# Autodesk Inventor assembly: 0005-10-04 Y axis and extruder
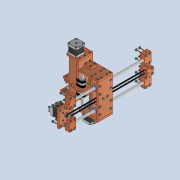
[picture p0: Inventor's stored thumbnail of the model, 180x180]
Saved by Autodesk Inventor 2020 (Build 240168000, 168)
## iProperties
Created: 2020-12-18
Part Number: 0005-10-04 Y axis and extruder
Document SubType Name: Assembly
Designer: Iulian Bors
Mass: 17144.8 g
Surface Area: 27601.7 cm^2
Volume: 16303.9 cm^3
Density: 1.05157 g/cm^3
Author: Iulian Bors
## iProperties of the stored document Part 1.ipt
Created: 2020-12-18
Part Number: Part 1
Material: Generic
Document SubType Name: Modeling
Designer: Iulian Bors
Density: 1 g/cm^3
Appearance: Default
Mass: 0.27605 g
Surface Area: 6.48852 cm^2
Volume: 0.27605 cm^3
Author: Iulian Bors
Revision Number: NONE
## iProperties of the stored document Part 2.ipt
Created: 2020-12-18
Part Number: Part 2
Material: Generic
Document SubType Name: Modeling
Designer: Iulian Bors
Density: 1 g/cm^3
Appearance: Default
Mass: 0.0253291 g
Surface Area: 2.0565 cm^2
Volume: 0.0253291 cm^3
Author: Iulian Bors
Revision Number: NONE
## iProperties of the stored document Needle.iam
Created: 2020-01-23
Part Number: Needle
Document SubType Name: Assembly
Designer: Iulian Bors
Mass: 0.301379 g
Surface Area: 8.54503 cm^2
Volume: 0.301379 cm^3
Density: 1 g/cm^3
Title: /vol/tmp/translate-4006329005178005204/5e293bbb2de6b7156cc2e2d4.step
## Documents named in this file (37)
- Z:\I.A.B\Proiecte\0005 I.A.B 3d 2.0 Imprimanta aracet\10 Mecanic\0005-10-04 Y axis and extruder.iam
- Z:\I.A.B\Proiecte\0005 I.A.B 3d 2.0 Imprimanta aracet\10 Mecanic\Seringa\body 20ml_Défaut.ipt
- Z:\I.A.B\Proiecte\0005 I.A.B 3d 2.0 Imprimanta aracet\10 Mecanic\Seringa\Plunger Assembly_Défaut.iam
- **Z:\I.A.B\Proiecte\0005 I.A.B 3d 2.0 Imprimanta aracet\10 Mecanic\0005-10-04 Y axis and extruder.iam*LocalDocs*xAaaaqeaaAaaaaaaaAaaaq3zaLd*Needle.iam
- Z:\I.A.B\Proiecte\0005 I.A.B 3d 2.0 Imprimanta aracet\10 Mecanic\0005-10-003 Actionare seringa.ipt
- Z:\I.A.B\Proiecte\0005 I.A.B 3d 2.0 Imprimanta aracet\10 Mecanic\0005-10-004 Actionare 2 seringa.ipt
- Z:\I.A.B\Proiecte\0005 I.A.B 3d 2.0 Imprimanta aracet\10 Mecanic\0005-10-1004 Piulita.ipt
- Z:\I.A.B\Proiecte\0005 I.A.B 3d 2.0 Imprimanta aracet\10 Mecanic\0005-10-10-1003 LeadScrew 8mm x 2mmPitch.ipt
- Z:\I.A.B\Proiecte\0005 I.A.B 3d 2.0 Imprimanta aracet\10 Mecanic\0005-10-1005 ISO 1224-1 - 10 - 8 x 22 x 7.ipt
- Z:\I.A.B\Proiecte\0005 I.A.B 3d 2.0 Imprimanta aracet\10 Mecanic\0005-10-005.ipt
- Z:\I.A.B\Proiecte\0005 I.A.B 3d 2.0 Imprimanta aracet\10 Mecanic\0005-10-006 Capac rulment.ipt
- Z:\I.A.B\Proiecte\0005 I.A.B 3d 2.0 Imprimanta aracet\10 Mecanic\0005-10-1002  Hub.ipt
- Z:\I.A.B\Proiecte\0005 I.A.B 3d 2.0 Imprimanta aracet\10 Mecanic\0005-10-1001 NEMA17 - Motor de passo.ipt
- Z:\I.A.B\Proiecte\0005 I.A.B 3d 2.0 Imprimanta aracet\10 Mecanic\0005-10-007Suport nema.ipt
- Z:\I.A.B\Proiecte\0005 I.A.B 3d 2.0 Imprimanta aracet\10 Mecanic\0005-10-008.ipt
- Z:\I.A.B\Proiecte\0005 I.A.B 3d 2.0 Imprimanta aracet\10 Mecanic\0005-10-009.ipt
- Z:\I.A.B\Proiecte\0005 I.A.B 3d 2.0 Imprimanta aracet\10 Mecanic\0005-10-010.ipt
- Z:\I.A.B\Proiecte\0005 I.A.B 3d 2.0 Imprimanta aracet\10 Mecanic\0005-10-1006 Bara rectificata.ipt
- Z:\I.A.B\Proiecte\0005 I.A.B 3d 2.0 Imprimanta aracet\10 Mecanic\0005-10-1009 LM10uu.ipt
- Z:\I.A.B\Proiecte\0005 I.A.B 3d 2.0 Imprimanta aracet\10 Mecanic\0005-10-002 Suport1 Seringa.ipt
- Z:\I.A.B\Proiecte\0005 I.A.B 3d 2.0 Imprimanta aracet\10 Mecanic\0005-10-016.ipt
- Z:\I.A.B\Proiecte\0005 I.A.B 3d 2.0 Imprimanta aracet\10 Mecanic\0005-10-021 suport senzor z.ipt
- Z:\I.A.B\Proiecte\0005 I.A.B 3d 2.0 Imprimanta aracet\10 Mecanic\0005-10-1000 LM8.ipt
- Z:\I.A.B\Proiecte\0005 I.A.B 3d 2.0 Imprimanta aracet\10 Mecanic\0005-10-1018 tija 8.ipt
- Z:\I.A.B\Proiecte\0005 I.A.B 3d 2.0 Imprimanta aracet\10 Mecanic\Surub M3 40 mm.iam
- Z:\I.A.B\Proiecte\0005 I.A.B 3d 2.0 Imprimanta aracet\10 Mecanic\0005-10-1020 ISO 7089 - 3 - 140 HV(1).ipt
- Z:\I.A.B\Proiecte\0005 I.A.B 3d 2.0 Imprimanta aracet\10 Mecanic\0005-10-01 Cadru.iam
- Z:\I.A.B\Proiecte\0005 I.A.B 3d 2.0 Imprimanta aracet\10 Mecanic\0005-10-02 X axis.iam
- Z:\I.A.B\Proiecte\0005 I.A.B 3d 2.0 Imprimanta aracet\10 Mecanic\0005-10-1032.ipt
- Z:\I.A.B\Proiecte\0005 I.A.B 3d 2.0 Imprimanta aracet\10 Mecanic\Surub M3 25.iam
- Z:\I.A.B\Proiecte\0005 I.A.B 3d 2.0 Imprimanta aracet\10 Mecanic\0005-10-1021 ISO 4032 - M3 - ISO.ipt
- Z:\I.A.B\Proiecte\0005 I.A.B 3d 2.0 Imprimanta aracet\10 Mecanic\Colier.ipt
- C:\Users\40743\Documents\Inventor\Content Center Files\R2020\en-US\ISO 7050 - C-Z(2)\ISO 7050 - ST 3.5 x 22 - C - Z.ipt
- **Z:\I.A.B\Proiecte\0005 I.A.B 3d 2.0 Imprimanta aracet\0005-00-00 Ansamblu_General.iam*LocalDocs*xAaaaaecaAaaaaaaaAaaaqfy1Od*Part 1.ipt
- **Z:\I.A.B\Proiecte\0005 I.A.B 3d 2.0 Imprimanta aracet\0005-00-00 Ansamblu_General.iam*LocalDocs*xAaaaa4baAaaaaaaaAaaaq4bsZa*Part 2.ipt
- **Z:\I.A.B\Proiecte\0005 I.A.B 3d 2.0 Imprimanta aracet\0005-00-00 Ansamblu_General.iam*LocalDocs*xAaaaqeaaAaaaaaaaAaaaq3zaLd*Needle.iam
- Z:\I.A.B\Proiecte\0005 I.A.B 3d 2.0 Imprimanta aracet\10 Mecanic\Seringa\21-gauge-needle-1.snapshot.2\Needle.step
## Components (93 placed, 33 different names)
1. Needle.iam:4 [sub-assembly] — Insert:14
2. 0005-10-10-1003 LeadScrew 8mm x 2mmPitch.ipt:5 — Insert:2, Insert:4, Mate:61, Mate:118
3. 0005-10-1005 ISO 1224-1 - 10 - 8 x 22 x 7.ipt:6 — Insert:2, Mate:15, Insert:3
4. 0005-10-005.ipt:7 — Mate:15, Mate:16, Flush:4, Mate:17, Flush:76, Flush:7, Mate:50, Mate:51, Angle:9, Mate:59, Mate:61, Flush:35, Mate:137, Mate:138, Mate:142, Insert:67, Insert:68, Insert:76, Insert:77, Insert:78
5. 0005-10-006 Capac rulment.ipt:8 — Insert:3, Insert:62, Insert:63, Insert:64, Mate:142, Mate:143
6. 0005-10-1002  Hub.ipt:9 — Insert:4, Insert:5
7. 0005-10-1001 NEMA17 - Motor de passo.ipt:10 — Insert:5, Angle:14
8. 0005-10-008.ipt:11 — Mate:16, Flush:4, Flush:11, Mate:21, Angle:11, Mate:158, Mate:159
9. 0005-10-008.ipt:12 — Mate:17, Flush:7, Mate:119, Flush:64, Angle:16, Mate:157
10. 0005-10-016.ipt:13 — Flush:76, Mate:19, Mate:20, Flush:18, Flush:35, Flush:63
11. 0005-10-009.ipt:14 — Mate:19, Flush:11, Flush:18, Flush:63, Flush:65, Angle:15, Mate:157, Mate:158
12. 0005-10-010.ipt:15 — Mate:20, Mate:21, Insert:7, Mate:35, Mate:37, Mate:103, Insert:26, Insert:27, Mate:147, Mate:150, Mate:153, Mate:155, Mate:159
13. 0005-10-1004 Piulita.ipt:16 — Mate:35, Mate:36
14. 0005-10-1009 LM10uu.ipt:17 — Insert:7, Mate:26, Flush:57, Mate:145, Mate:146
15. 0005-10-1006 Bara rectificata.ipt:18 — Mate:26, Insert:41
16. 0005-10-1006 Bara rectificata.ipt:19 — Mate:103, Mate:104, Insert:42
17. 0005-10-10-1003 LeadScrew 8mm x 2mmPitch.ipt:21 — Mate:33, Mate:36, Mate:37, Insert:37, Insert:38
18. 0005-10-1002  Hub.ipt:22 — Mate:33
19. 0005-10-1001 NEMA17 - Motor de passo.ipt:23 — Insert:37, Mate:139, Angle:13
20. 0005-10-006 Capac rulment.ipt:26 — Insert:39, Mate:141
21. 0005-10-1005 ISO 1224-1 - 10 - 8 x 22 x 7.ipt:27 — Insert:38, Insert:39
22. 0005-10-1004 Piulita.ipt:38 — Insert:13, Mate:140, Insert:72
23. body 20ml_Défaut.ipt:39 — Mate:50, Mate:51, Angle:9, Mate:52, Insert:14
24. Plunger Assembly_Défaut.iam:40 [sub-assembly] — Mate:52, Mate:53
25. 0005-10-003 Actionare seringa.ipt:41 — Insert:13, Mate:53, Angle:11, Mate:117, Mate:118, Insert:22, Mate:121, Mate:122, Mate:140, Insert:65, Insert:66
26. 0005-10-004 Actionare 2 seringa.ipt:42 — Insert:22, Mate:122
27. 0005-10-002 Suport1 Seringa.ipt:43 — Mate:59, Mate:137, Mate:138
28. 0005-10-021 suport senzor z.ipt:75 — Mate:144
29. 0005-10-1009 LM10uu.ipt:79 — Mate:104, Flush:57, Mate:151, Flush:71, Mate:152
30. 0005-10-1000 LM8.ipt:85 — Mate:117, Mate:120
31. 0005-10-007Suport nema.ipt:86 — Mate:119, Flush:64, Flush:65, Flush:66, Angle:14, Insert:55, Insert:56, Insert:57, Insert:73, Insert:74, Insert:75
32. 0005-10-1018 tija 8.ipt:87 — Mate:120, Mate:121, Flush:66
33. Surub M3 40 mm.iam:89 [sub-assembly] — Insert:43
34. 0005-10-1009 LM10uu.ipt:91 — Insert:27, Mate:148, Flush:68, Mate:149
35. 0005-10-1009 LM10uu.ipt:92 — Insert:26, Mate:154, Mate:156, Flush:74
36. 0005-10-01 Cadru:1 [sub-assembly] — Insert:40
37. 0005-10-02 X axis:1 [sub-assembly] — Insert:40, Angle:12, Insert:41, Insert:42, Mate:139, Angle:13, Insert:43, Mate:141, Insert:44, Insert:45, Insert:46, Insert:58, Insert:59, Insert:60, Insert:61, Mate:144
38. Surub M3 40 mm:2 [sub-assembly] — Insert:44
39. Surub M3 40 mm:3 [sub-assembly] — Insert:45
40. Surub M3 40 mm:4 [sub-assembly] — Insert:46
41. DIN 7984 M3 x 16:1
42. ISO 7089 3:2 — Insert:55
43. DIN 7984 M3 x 16:2
44. ISO 7089 3:3 — Insert:58
45. DIN 7984 M3 x 16:4
46. ISO 7089 3:5 — Insert:57
47. DIN 7984 M3 x 16:5
48. ISO 7089 3:6 — Insert:61
49. DIN 7984 M3 x 16:6
50. ISO 7089 3:7 — Insert:59
51. DIN 7984 M3 x 16:7
52. ISO 7089 3:8 — Insert:60
53. DIN 7984 M3 x 16:8
54. ISO 7089 3:9 — Insert:56
55. Surub M3 40 mm:5 [sub-assembly] — Insert:64
56. Surub M3 40 mm:6 [sub-assembly] — Insert:63
57. Surub M3 40 mm:7 [sub-assembly] — Insert:62
58. Surub M3 40 mm:8 [sub-assembly] — Mate:143
59. Surub M3 25:1 [sub-assembly] — Insert:65
60. Surub M3 25:2 [sub-assembly] — Insert:66
61. Surub M3 25:3 [sub-assembly] — Insert:67
62. Surub M3 25:4 [sub-assembly] — Insert:68
63. Colier:1 — Mate:145, Angle:15, Flush:67
64. Colier:2 — Mate:146, Mate:147, Flush:67, Flush:69, Flush:70
65. Colier:3 — Mate:148, Flush:68, Flush:69
66. Colier:4 — Mate:149, Mate:150, Flush:70
67. Colier:5 — Mate:151, Angle:16, Flush:71, Flush:72
68. Colier:6 — Mate:152, Mate:153, Flush:72, Flush:73
69. Colier:7 — Mate:154, Mate:155, Flush:73, Flush:75
70. Colier:8 — Mate:156, Flush:74, Flush:75
71. ISO 7050 - C-Z ST 3.5 x 22 - C - Z:1 — Insert:73
72. ISO 7050 - C-Z ST 3.5 x 22 - C - Z:2 — Insert:76
73. ISO 7050 - C-Z ST 3.5 x 22 - C - Z:3 — Insert:78
74. ISO 7050 - C-Z ST 3.5 x 22 - C - Z:4 — Insert:74
75. ISO 7050 - C-Z ST 3.5 x 22 - C - Z:5 — Insert:75
76. ISO 7050 - C-Z ST 3.5 x 22 - C - Z:6 — Insert:77
77. ISO 7050 - C-Z ST 3.5 x 22 - C - Z:7
78. DIN 7984 M3 x 16:9 — Insert:70
79. ISO 7089 3:10 — Insert:72
80. ISO 4032 M3:1 — Insert:70, Insert:71
81. ISO 7089 3:11 — Insert:71
82. DIN 7984 M3 x 16:10
83. ISO 7089 3:12
84. ISO 4032 M3:2
85. ISO 7089 3:13
86. DIN 7984 M3 x 16:11
87. ISO 7089 3:14
88. ISO 4032 M3:3
89. ISO 7089 3:15
90. DIN 7984 M3 x 16:12
91. ISO 7089 3:16
92. ISO 4032 M3:4
93. ISO 7089 3:17
## Component patterns: (4 elements, first: DIN 7984 M3 x 16:9 + ISO 7089 3:10 + ISO 4032 M3:1 + ISO 7089 3:11)
## Relationships (127: Insert 52, Mate 48, Flush 20, Angle 7)
- Insert:2: 0005-10-10-1003 LeadScrew 8mm x 2mmPitch.ipt:5 ↔ 0005-10-1005 ISO 1224-1 - 10 - 8 x 22 x 7.ipt:6
- Mate:15: 0005-10-1005 ISO 1224-1 - 10 - 8 x 22 x 7.ipt:6 ↔ 0005-10-005.ipt:7
- Insert:3: 0005-10-1005 ISO 1224-1 - 10 - 8 x 22 x 7.ipt:6 ↔ 0005-10-006 Capac rulment.ipt:8
- Insert:4: 0005-10-10-1003 LeadScrew 8mm x 2mmPitch.ipt:5 ↔ 0005-10-1002  Hub.ipt:9
- Insert:5 (5 mm): 0005-10-1002  Hub.ipt:9 ↔ 0005-10-1001 NEMA17 - Motor de passo.ipt:10
- Mate:16: 0005-10-005.ipt:7 ↔ 0005-10-008.ipt:11
- Flush:4: 0005-10-005.ipt:7 ↔ 0005-10-008.ipt:11
- Mate:17: 0005-10-005.ipt:7 ↔ 0005-10-008.ipt:12
- Flush:76: 0005-10-005.ipt:7 ↔ 0005-10-016.ipt:13
- Flush:7: 0005-10-005.ipt:7 ↔ 0005-10-008.ipt:12
- Mate:19 (8 mm): 0005-10-016.ipt:13 ↔ 0005-10-009.ipt:14
- Flush:11: 0005-10-008.ipt:11 ↔ 0005-10-009.ipt:14
- Mate:20: 0005-10-016.ipt:13 ↔ 0005-10-010.ipt:15
- Mate:21: 0005-10-008.ipt:11 ↔ 0005-10-010.ipt:15
- Insert:7: 0005-10-010.ipt:15 ↔ 0005-10-1009 LM10uu.ipt:17
- Mate:26: 0005-10-1009 LM10uu.ipt:17 ↔ 0005-10-1006 Bara rectificata.ipt:18
- [Insert] (5 mm): 0005-10-1002  Hub.ipt:22 ↔ 0005-10-1001 NEMA17 - Motor de passo.ipt:23
- Mate:33: 0005-10-10-1003 LeadScrew 8mm x 2mmPitch.ipt:21 ↔ 0005-10-1002  Hub.ipt:22
- Mate:35: 0005-10-010.ipt:15 ↔ 0005-10-1004 Piulita.ipt:16
- Mate:36: 0005-10-1004 Piulita.ipt:16 ↔ 0005-10-10-1003 LeadScrew 8mm x 2mmPitch.ipt:21
- Mate:37: 0005-10-010.ipt:15 ↔ 0005-10-10-1003 LeadScrew 8mm x 2mmPitch.ipt:21
- Flush:18: 0005-10-016.ipt:13 ↔ 0005-10-009.ipt:14
- Mate:50: 0005-10-005.ipt:7 ↔ body 20ml_Défaut.ipt:39
- Mate:51: 0005-10-005.ipt:7 ↔ body 20ml_Défaut.ipt:39
- Angle:9 (0 deg): 0005-10-005.ipt:7 ↔ body 20ml_Défaut.ipt:39
- Mate:52: body 20ml_Défaut.ipt:39 ↔ Plunger Assembly_Défaut.iam:40
- Insert:13: 0005-10-1004 Piulita.ipt:38 ↔ 0005-10-003 Actionare seringa.ipt:41
- Mate:53: Plunger Assembly_Défaut.iam:40 ↔ 0005-10-003 Actionare seringa.ipt:41
- Insert:14 (-5 mm): Needle.iam:4 ↔ body 20ml_Défaut.ipt:39
- Angle:11 (0 deg): 0005-10-008.ipt:11 ↔ 0005-10-003 Actionare seringa.ipt:41
- Mate:59: 0005-10-005.ipt:7 ↔ 0005-10-002 Suport1 Seringa.ipt:43
- Mate:61: 0005-10-10-1003 LeadScrew 8mm x 2mmPitch.ipt:5 ↔ 0005-10-005.ipt:7
- Flush:35 (8 mm): 0005-10-005.ipt:7 ↔ 0005-10-016.ipt:13
- Mate:103: 0005-10-010.ipt:15 ↔ 0005-10-1006 Bara rectificata.ipt:19
- Mate:104: 0005-10-1006 Bara rectificata.ipt:19 ↔ 0005-10-1009 LM10uu.ipt:79
- Flush:57: 0005-10-1009 LM10uu.ipt:17 ↔ 0005-10-1009 LM10uu.ipt:79
- Mate:117 (-10 mm): 0005-10-003 Actionare seringa.ipt:41 ↔ 0005-10-1000 LM8.ipt:85
- Mate:118: 0005-10-10-1003 LeadScrew 8mm x 2mmPitch.ipt:5 ↔ 0005-10-003 Actionare seringa.ipt:41
- Flush:63: 0005-10-016.ipt:13 ↔ 0005-10-009.ipt:14
- Insert:22 (1 mm): 0005-10-003 Actionare seringa.ipt:41 ↔ 0005-10-004 Actionare 2 seringa.ipt:42
- Mate:119: 0005-10-008.ipt:12 ↔ 0005-10-007Suport nema.ipt:86
- Flush:64: 0005-10-008.ipt:12 ↔ 0005-10-007Suport nema.ipt:86
- Flush:65: 0005-10-009.ipt:14 ↔ 0005-10-007Suport nema.ipt:86
- Mate:120: 0005-10-1000 LM8.ipt:85 ↔ 0005-10-1018 tija 8.ipt:87
- Mate:121: 0005-10-003 Actionare seringa.ipt:41 ↔ 0005-10-1018 tija 8.ipt:87
- Flush:66: 0005-10-007Suport nema.ipt:86 ↔ 0005-10-1018 tija 8.ipt:87
- Mate:122: 0005-10-003 Actionare seringa.ipt:41 ↔ 0005-10-004 Actionare 2 seringa.ipt:42
- Insert:26: 0005-10-010.ipt:15 ↔ 0005-10-1009 LM10uu.ipt:92
- Insert:27: 0005-10-010.ipt:15 ↔ 0005-10-1009 LM10uu.ipt:91
- Mate:137: 0005-10-005.ipt:7 ↔ 0005-10-002 Suport1 Seringa.ipt:43
- Mate:138: 0005-10-005.ipt:7 ↔ 0005-10-002 Suport1 Seringa.ipt:43
- Insert:37: 0005-10-10-1003 LeadScrew 8mm x 2mmPitch.ipt:21 ↔ 0005-10-1001 NEMA17 - Motor de passo.ipt:23
- Insert:38: 0005-10-10-1003 LeadScrew 8mm x 2mmPitch.ipt:21 ↔ 0005-10-1005 ISO 1224-1 - 10 - 8 x 22 x 7.ipt:27
- Insert:39: 0005-10-006 Capac rulment.ipt:26 ↔ 0005-10-1005 ISO 1224-1 - 10 - 8 x 22 x 7.ipt:27
- Insert:40: 0005-10-01 Cadru:1 ↔ 0005-10-02 X axis:1
- Angle:12 (0 deg): 0005-10-02 X axis:1
- Insert:41: 0005-10-1006 Bara rectificata.ipt:18 ↔ 0005-10-02 X axis:1
- Insert:42: 0005-10-1006 Bara rectificata.ipt:19 ↔ 0005-10-02 X axis:1
- Mate:139: 0005-10-1001 NEMA17 - Motor de passo.ipt:23 ↔ 0005-10-02 X axis:1
- Angle:13 (0 deg): 0005-10-1001 NEMA17 - Motor de passo.ipt:23 ↔ 0005-10-02 X axis:1
- Angle:14 (0 deg): 0005-10-1001 NEMA17 - Motor de passo.ipt:10 ↔ 0005-10-007Suport nema.ipt:86
- Mate:140: 0005-10-1004 Piulita.ipt:38 ↔ 0005-10-003 Actionare seringa.ipt:41
- Insert:43: Surub M3 40 mm.iam:89 ↔ 0005-10-02 X axis:1
- Mate:141: 0005-10-006 Capac rulment.ipt:26 ↔ 0005-10-02 X axis:1
- Insert:44: 0005-10-02 X axis:1 ↔ Surub M3 40 mm:2
- Insert:45: 0005-10-02 X axis:1 ↔ Surub M3 40 mm:3
- Insert:46: 0005-10-02 X axis:1 ↔ Surub M3 40 mm:4
- [Insert]: DIN 7984 M3 x 16:1 ↔ ISO 7089 3:2
- [Insert]: DIN 7984 M3 x 16:2 ↔ ISO 7089 3:3
- [Insert]: DIN 7984 M3 x 16:4 ↔ ISO 7089 3:5
- [Insert]: DIN 7984 M3 x 16:5 ↔ ISO 7089 3:6
- [Insert]: DIN 7984 M3 x 16:6 ↔ ISO 7089 3:7
- [Insert]: DIN 7984 M3 x 16:7 ↔ ISO 7089 3:8
- [Insert]: DIN 7984 M3 x 16:8 ↔ ISO 7089 3:9
- Insert:55: 0005-10-007Suport nema.ipt:86 ↔ ISO 7089 3:2
- Insert:56: 0005-10-007Suport nema.ipt:86 ↔ ISO 7089 3:9
- Insert:57: 0005-10-007Suport nema.ipt:86 ↔ ISO 7089 3:5
- Insert:58: 0005-10-02 X axis:1 ↔ ISO 7089 3:3
- Insert:59: 0005-10-02 X axis:1 ↔ ISO 7089 3:7
- Insert:60: 0005-10-02 X axis:1 ↔ ISO 7089 3:8
- Insert:61: 0005-10-02 X axis:1 ↔ ISO 7089 3:6
- Insert:62: 0005-10-006 Capac rulment.ipt:8 ↔ Surub M3 40 mm:7
- Insert:63: 0005-10-006 Capac rulment.ipt:8 ↔ Surub M3 40 mm:6
- Insert:64: 0005-10-006 Capac rulment.ipt:8 ↔ Surub M3 40 mm:5
- Mate:142: 0005-10-005.ipt:7 ↔ 0005-10-006 Capac rulment.ipt:8
- Mate:143: 0005-10-006 Capac rulment.ipt:8 ↔ Surub M3 40 mm:8
- Insert:65: 0005-10-003 Actionare seringa.ipt:41 ↔ Surub M3 25:1
- Insert:66: 0005-10-003 Actionare seringa.ipt:41 ↔ Surub M3 25:2
- Insert:67: 0005-10-005.ipt:7 ↔ Surub M3 25:3
- Insert:68: 0005-10-005.ipt:7 ↔ Surub M3 25:4
- Mate:144: 0005-10-021 suport senzor z.ipt:75 ↔ 0005-10-02 X axis:1
- [Insert]: DIN 7984 M3 x 16:9 ↔ ISO 7089 3:10
- Insert:70: DIN 7984 M3 x 16:9 ↔ ISO 4032 M3:1
- Insert:71: ISO 4032 M3:1 ↔ ISO 7089 3:11
- Insert:72: 0005-10-1004 Piulita.ipt:38 ↔ ISO 7089 3:10
- Mate:145: 0005-10-1009 LM10uu.ipt:17 ↔ Colier:1
- Angle:15 (180 deg): 0005-10-009.ipt:14 ↔ Colier:1
- Mate:146: 0005-10-1009 LM10uu.ipt:17 ↔ Colier:2
- Mate:147: 0005-10-010.ipt:15 ↔ Colier:2
- Flush:67: Colier:1 ↔ Colier:2
- Mate:148: 0005-10-1009 LM10uu.ipt:91 ↔ Colier:3
- Flush:68: 0005-10-1009 LM10uu.ipt:91 ↔ Colier:3
- Flush:69: Colier:2 ↔ Colier:3
- Mate:149: 0005-10-1009 LM10uu.ipt:91 ↔ Colier:4
- Mate:150: 0005-10-010.ipt:15 ↔ Colier:4
- Flush:70: Colier:2 ↔ Colier:4
- Mate:151: 0005-10-1009 LM10uu.ipt:79 ↔ Colier:5
- Angle:16 (0 deg): 0005-10-008.ipt:12 ↔ Colier:5
- Flush:71: 0005-10-1009 LM10uu.ipt:79 ↔ Colier:5
- Mate:152: 0005-10-1009 LM10uu.ipt:79 ↔ Colier:6
- Mate:153: 0005-10-010.ipt:15 ↔ Colier:6
- Flush:72: Colier:5 ↔ Colier:6
- Mate:154: 0005-10-1009 LM10uu.ipt:92 ↔ Colier:7
- Mate:155: 0005-10-010.ipt:15 ↔ Colier:7
- Flush:73: Colier:6 ↔ Colier:7
- Mate:156: 0005-10-1009 LM10uu.ipt:92 ↔ Colier:8
- Flush:74: 0005-10-1009 LM10uu.ipt:92 ↔ Colier:8
- Flush:75: Colier:7 ↔ Colier:8
- Mate:157: 0005-10-008.ipt:12 ↔ 0005-10-009.ipt:14
- Mate:158: 0005-10-008.ipt:11 ↔ 0005-10-009.ipt:14
- Mate:159: 0005-10-008.ipt:11 ↔ 0005-10-010.ipt:15
- Insert:73: 0005-10-007Suport nema.ipt:86 ↔ ISO 7050 - C-Z ST 3.5 x 22 - C - Z:1
- Insert:74: 0005-10-007Suport nema.ipt:86 ↔ ISO 7050 - C-Z ST 3.5 x 22 - C - Z:4
- Insert:75: 0005-10-007Suport nema.ipt:86 ↔ ISO 7050 - C-Z ST 3.5 x 22 - C - Z:5
- Insert:76: 0005-10-005.ipt:7 ↔ ISO 7050 - C-Z ST 3.5 x 22 - C - Z:2
- Insert:77: 0005-10-005.ipt:7 ↔ ISO 7050 - C-Z ST 3.5 x 22 - C - Z:6
- Insert:78: 0005-10-005.ipt:7 ↔ ISO 7050 - C-Z ST 3.5 x 22 - C - Z:3
## Named parameters: d64_d31 = 5 mm, d387_d441 = 0 mm, d389_d441 = 0 mm, d390_d441 = 0 mm, d391_d441 = 0 mm, d392_d441 = 0 mm, d393_d441 = 0 mm, d412_d390_d441 = 0 mm
